# Autodesk Inventor assembly: 043.5-DXP(F,D-166-3)
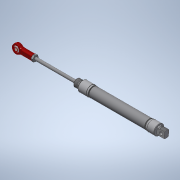
[picture p0: Inventor's stored thumbnail of the model, 180x180]
Saved by Autodesk Inventor 2020 (Build 240168000, 168)
## iProperties
Created: 2019-01-26
Part Number: 043.5-DXP(F,D-166-3)
Catalog Web Link: www.cadenas.de
Description: Original Line Standard Air Cylinders-Standard Air Cylinders
Vendor: BIMBA
Document SubType Name: Assembly
Designer: psadmin
Manufacturer: BIMBA
Mass: 155.922 g
Surface Area: 318.239 cm^2
Volume: 38.1991 cm^3
Density: 4.08184 g/cm^3
Category: PARTsolutions
Company: BIMBA
PSOL_IDENT_0: {$CADENAS_DATA\23d-libs\bimba\bimba\bimba_imperial\bimba_full_line\original_line_cylinders\standard_
PSOL_IDENT_1: air_cylinders\standard_air_cylinder_asmtab.prj},337 {VTYP=3D},{STYP=ASSTAB},{NB=043.5-DXP(F,D-166-3)
PSOL_IDENT_2: },{LINA=043.5-DXP},{NN=Original Line Standard Air Cylinders},{DATE=21.03.2018 14:31:21},{GEOMDATE=19
PSOL_IDENT_3: .03.2018 11:39:15},{VERSION=},{LINEID=50},{WBVAR=STROKE,ACTING,MNT,DER,NR,BM,CO,OO,VO,M,EE,EEL,K,Q,Y
PSOL_IDENT_4: ,G,T,HL,B,H,SER,SR,NT,W,STPT1,STPT2,STPT3,STPT4,MB,PB,PRC,TB,MN},{WBNUMERIC=STROKE,EEL}  {NB=043.5-D
PSOL_IDENT_5: XP(F,D-166-3)},{LINA=043.5-DXP},{KT=DUMMY},{PN=043.5-DXP},{PNC=043.5-DXP(F,D-166-3)},{PNA=(D-166-3)}
PSOL_IDENT_6: ,{DASH=-},{BORE1=0.75000000},{BORE=3/4\" (04)},{BOREPN=04},{STROKE=3.500},{STROKEALG=[0.011:50/0.001
PSOL_IDENT_7: ]},{STROKE1=3.500},{ACTING=D},{ACTINGALG= '' , 'Single Acting (SA)' , 'R' , 'Reverse Single Acting (
PSOL_IDENT_8: SA)' , 'D' , 'Double Acting (SA)' },{ACTINGPN=D},{MNT=XP},{MNTALG= '' , 'Front Nose Mounting (SA)' ,
PSOL_IDENT_9: 'P' , 'Rear Pivot Mounting (SA)' , 'XP' , 'Double End or Pivot Mounting (SA)' , 'X' , 'Double End M
PSOL_IDENT_10: ounting (SA)' , 'BF' , 'Front Block Mounting (SA)' , 'BR' , 'Rear Block Mounting for Vertical Positi
PSOL_IDENT_11: oning (SA)' , 'BFT' , 'Front Block Trunnion Mounting (SA)' , 'BRT' , 'Rear Block Trunnion Mounting (
PSOL_IDENT_12: SA)' },{TYPE=},{MNTPN=XP},{DER=},{DERALG= '' , 'N/A' },{NR=},{NRALG= '' , 'N/A' },{NRPN=},{BM=},{BMA
PSOL_IDENT_13: LG= '' , 'N/A' },{BMPN=},{CO=},{COALG= '' , 'N/A' },{OO=},{OOALG= '', 'N/A' },{OOPN=},{VO=Z},{VOALG=
PSOL_IDENT_14: 'Z' , 'N/A' },{VOPN=},{OOVOPN=},{M=},{MALG= '', 'Without Magnet', 'M', 'With Magnet' },{EE=},{EEL=0
PSOL_IDENT_15: .000},{EEMAX=46.5000},{EEALG= '', 'Without Extra Extension', 'EE', 'With Extra Extension' },{EELALG=
PSOL_IDENT_16: 0},{EEPN=},{EEPN1=0.000},{K=},{KALG= '', 'Standard' , 'K' , 'Ports Rotated 90deg K' },{KPN=},{Q=},{Q
PSOL_IDENT_17: ALG= '' , 'N/A' },{QPN=},{Y=},{YALG= '' , 'Without Pivot Bushing' , 'Y' , 'With Pivot Bushing' },{YP
PSOL_IDENT_18: N=},{YCON=},{F=},{FALG= '', 'Non-Coated (Standard)', 'F', 'Molycoated' },{FPN=},{G=},{GPN=},{GPN99=}
PSOL_IDENT_19: ,{T=},{TALG= '' , 'Standard -20° to 200°F (-29° to 95°C)' , 'N' , 'Low Temperature' , 'V' , 'High Te
PSOL_IDENT_20: mperature' },{NPN=},{VPN=},{HL=},{HLALG= '' , 'Without Low Pressure Hydraulic' , 'HL' , 'With Low Pr
PSOL_IDENT_21: essure Hydraulic' },{B=},{BALG= '', 'W/out Bumpers' , 'B' , 'W/ Bumpers' },{BPN=},{H=},{HALG= '', 'N
PSOL_IDENT_22: /A' },{HPN=},{SER=},{SERALG= '' , 'Without Spring Extend/Return' , 'JS' , 'With Spring Return' , 'JR'
PSOL_IDENT_23: , 'With Spring Extend' },{SR=},{SRALG= '' , 'Standard Stainless Steel' },{SRPN=},{SRCON=0},{NT=},{N
PSOL_IDENT_24: TPN=},{W=},{WALG= '' , 'Without Wiper' , 'W' , 'With Wiper' },{WPN=},{E=},{EALG= '' , 'Standard Seal
PSOL_IDENT_25: s/Lube' , 'E' , 'Non-Lube Seals/Lube' },{EPN=},{ST=},{STALG= '' , 'N/A' },{STPT1=},{STPT1ALG= '' , '
PSOL_IDENT_26: N/A' },{STPT2=},{STPT2ALG= '' , 'N/A' },{STPT3=},{STPT3ALG= '' , 'N/A' },{STPT4=},{STPT4ALG= '' , 'N
PSOL_IDENT_27: /A' },{STPN=},{MB=},{MBALG= '' , 'Without Mounting Bracket' , 'F,D-129' , 'D-129 (front)'  , 'R,D-12
PSOL_IDENT_28: 9' , 'D-129 (rear)' , '2x,D-129' , 'D-129 (front & rear)'},{MBPN=},{MBPNALL=D-129},{MBPNALLREAR=D-12
PSOL_IDENT_29: 9},{PB=},{PBALG= '' , 'Without Pivot Bracket' , 'D-13498-A' , 'D-13498-A' },{PBPN=},{PBPNALL=D-13498
PSOL_IDENT_30: -A},{PRC=F,D-166-3},{PRCALG= '' , 'W/out Pivot Rod Clevis' , 'F,D-166-3' , 'D-166-3 (front)' },{PRCP
PSOL_IDENT_31: N=(F,D-166-3)},{PRCPNALL=D-166-3},{TB=},{TBALG= '' , 'N/A' },{TBPN=},{TBPNALL=},{MN=},{MNALG= '' , '
PSOL_IDENT_32: N/A' },{MNPN=},{MNCONF=},{MNCONR=},{TLEN=4.7555},{FRAC=17.2500},{RGCON=},{RGDACCON=R},{RHCON=P},{RHC
PSOL_IDENT_33: ON1=P},{RHCONON=1},{RHACCON=},{FNUTCON=1},{RNUTCON=1},{FNUTPN=D-9},{RNUTPN=D-9},{FNUTTRANS=0.0000},{
PSOL_IDENT_34: RNUTTRANS=0.0000},{VHOLECON=0},{A1=1.5940},{A1N=0.8750},{A1P=1.5940},{A1B=1.5940},{A4=0.2525},{A4N=0
PSOL_IDENT_35: .3130},{A4P=0.2525},{A5=0.0300},{A1H=1.594},{A1NH=0.5310},{A1PH=1.5940},{A1BH=1.0940},{A1SH=1.2190},
PSOL_IDENT_36: {A2H=0.2190},{A2NH=0.2190},{LENGTH=3.7500},{LENGTH1=3.7500},{LENGTH2=3.8100},{MUL=3.5000},{MUL11=3.5
PSOL_IDENT_37: 000},{MUL22=9.415},{MUL33=5.9150},{MUL2=3.5000},{MUL211=3.5000},{MUL222=2.6900},{MUL233=1.6900},{SSS=
PSOL_IDENT_38: 7.0000},{RGLEN=1.3715},{RHLEN=1.1230},{SSS1=4.0000},{A13=1.3120},{DIF=0.0000},{G5=0.6250},{ON=0},{SS
PSOL_IDENT_39: ADD=0.0000},{BADD=0.0000},{MADD=0.0000},{NVADD=0.0000},{TRACKL=4.4655},{TRACKCON=D-74168},{TRIMCON=0
PSOL_IDENT_40: },{TRIMCON1=0},{PINCON=D-51},{FSPACE=0.7247},{SPACE=0.0804},{TEXT=0.1406},{S1=1.0000},{D1=0.8325},{D
PSOL_IDENT_41: 1N=0.8050},{D1B=0.8625},{D1P=0.8325},{FA=0.940},{RA=0.9400},{PPATH=standard_air_cylinder_asmtpl.prj}
PSOL_IDENT_42: ,{MATALGHTML=<b>Standard Original Line:</b><dl><dt>Rod:</dt><dd>- Stainless Steel</dd><dd>&nbsp;&nbs
PSOL_IDENT_43: p;(5/16 9/16 Bores)</dd><dd>- High Strength Carbon Steel</dd><dd>&nbsp;&nbsp;(3/4 3 Bore)</dd><dd>-
PSOL_IDENT_44: Stainless Steel</dd><dd>&nbsp;&nbsp;(X style DXP/DX/DXDE)</dd><dt>Bearings:</dt><dd>- Sintered Bronz
PSOL_IDENT_45: e</dd><dt>Body:</dt><dd>- 304 Stainless Steel</dd><dt>End Caps:</dt><dd>- Aluminum</dd><dt>Seals:</d
PSOL_IDENT_46: t><dd>- Buna N</dd></dl>},{ASSCFGPRA=04DXP},{MBPNA=},{MNPNA=},{PRCPNA=(D-166-3)},{ASSOPTACC=STPT4},{
PSOL_IDENT_47: A=7.25},{HADD=0.0000},{WFL=0.25},{QADD=0.000},{QADD1=0.440},{TEST=3.0000},{MNTB=},{STDNUTF=1},{STDNU
PSOL_IDENT_48: TR=1},{STRK2D=0},{X2D=2},{STROKESW=3.500},{EESW=0.000},{FCD=0},{BCD=0},{RCD=0},{CUSTADD=2.500},{FT=1
PSOL_IDENT_49: /4-28 UNF-2A},{FT1=1/4-28 UNF-2A},{FT2=5/8-18 UNF-2A},{PORT=1/8 NPT},{FT11=1/2-20 UNF-2A},{FT12=5/8-
PSOL_IDENT_50: 18 UNF-2A},{B1=}
NN: Original Line Standard Air Cylinders
NT: Standard Male Thread
NB: 043.5-DXP(F,D-166-3)
NBSYN: $PNC.
LINA: 043.5-DXP
PN: 043.5-DXP
PNA: (D-166-3)
BORE: 3/4" (04)
STROKE: 3.5
ACTING: Double [D]
MNT: Universal Double End or Rear Pivot [XP]
DER: N/A
NR: N/A
BM: N/A
CO: N/A
OO: N/A
VO: N/A
M: Without Magnet Piston
EE: Standard Rod Extension
EEL: 0
K: Standard
Q: N/A
Y: Standard Pivot Style
G: Standard Grease Lube
T: Standard -20° to 200°F (-29° to 95°C)
HL: Standard 250 PSI Air
B: Without Bumpers
H: N/A
SER: Without Failsafe Spring Extend/Return
SR: Standard Stainless Steel
W: Without Wiper
STPT1: N/A
STPT2: N/A
STPT3: N/A
STPT4: N/A
MB: Without Mounting Bracket
PB: Without Pivot Bracket
PRC: D-166-3 (front)
TB: N/A
MN: N/A
A: 7.25
SUPPLIER: BIMBA
ARTICLENO: 043.5-DXP(F,D-166-3)
BOMINFO: 043.5-DXP
CREATOR: CADENAS GmbH
Title: 043.5-DXP
Author: Cadenas PARTsolutions
Comments: Standard Air Cylinders
## Documents named in this file (9)
- T:\EIT\2022 Rapid React\COMMON PARTS\AIR CYLINDERS\043.5-DXP\AIS2019\043_5-DXP(F,D-166-3).iam
- T:\EIT\2022 Rapid React\COMMON PARTS\AIR CYLINDERS\043.5-DXP\AIS2019\043_5-DXP(F,D-166-3)0000000_0_dummy.ipt
- T:\EIT\2022 Rapid React\COMMON PARTS\AIR CYLINDERS\043.5-DXP\AIS2019\04R000-0_rod_guide.ipt
- T:\EIT\2022 Rapid React\COMMON PARTS\AIR CYLINDERS\043.5-DXP\AIS2019\04R-4_75550.ipt
- T:\EIT\2022 Rapid React\COMMON PARTS\AIR CYLINDERS\043.5-DXP\AIS2019\04P0000_rear_head.ipt
- T:\EIT\2022 Rapid React\COMMON PARTS\AIR CYLINDERS\043.5-DXP\AIS2019\043_5-DXP0000_rod.ipt
- T:\EIT\2022 Rapid React\COMMON PARTS\AIR CYLINDERS\043.5-DXP\AIS2019\D-166-3-dummy.ipt
- T:\EIT\2022 Rapid React\COMMON PARTS\AIR CYLINDERS\043.5-DXP\AIS2019\D-344.ipt
- T:\EIT\2022 Rapid React\COMMON PARTS\AIR CYLINDERS\TieRod End\60685K321_PTFE-LINED ALUMINUM BALL JOINT ROD END.ipt
## Components (8 placed, 8 different names)
1. 043_5-DXP(F,D-166-3)0000000_0_dummy:1
2. 04R000-0_rod_guide:1 — Insert:1, Insert:4, Angle:2
3. 04R-4_75550:1 — Insert:1, Insert:2
4. 04P0000_rear_head:1 — Insert:2, Angle:1, Angle:2
5. 043_5-DXP0000_rod:1 — Insert:3, Insert:4
6. D-166-3-dummy:1
7. D-344:1 — Insert:3, Insert:5
8. 60685K321_PTFE-LINED ALUMINUM BALL JOINT ROD END:1 — Insert:5, Angle:1
## Relationships (7: Insert 5, Angle 2)
- Insert:1: 04R000-0_rod_guide:1 ↔ 04R-4_75550:1
- Insert:2: 04R-4_75550:1 ↔ 04P0000_rear_head:1
- Insert:3: 043_5-DXP0000_rod:1 ↔ D-344:1
- Insert:4: 04R000-0_rod_guide:1 ↔ 043_5-DXP0000_rod:1
- Insert:5 (0.762 mm): D-344:1 ↔ 60685K321_PTFE-LINED ALUMINUM BALL JOINT ROD END:1
- Angle:1 (0 deg): 04P0000_rear_head:1 ↔ 60685K321_PTFE-LINED ALUMINUM BALL JOINT ROD END:1
- Angle:2 (0 deg): 04R000-0_rod_guide:1 ↔ 04P0000_rear_head:1
